# Autodesk Inventor assembly: СБ_Лицевой лист
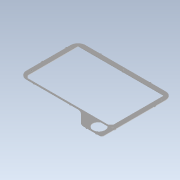
[picture p0: Inventor's stored thumbnail of the model, 180x180]
Saved by Autodesk Inventor 2021.2 (Build 252289000, 289)
## iProperties
Created: 2022-12-06
Part Number: СБ_Лицевой лист
Document SubType Name: Assembly
Designer: Королев В. В.
Mass: 46.2815 g
Surface Area: 491.583 cm^2
Volume: 42.8372 cm^3
Density: 1.0804 g/cm^3
Author: Королев В. В.
## Documents named in this file (3)
- C:\Users\Voodoo\Documents\Inventor\АБТ_Инфотабло\СБ_Лицевой лист.iam
- C:\Users\Voodoo\Documents\Inventor\АБТ_Инфотабло\Лицевой лист.ipt
- C:\Users\Voodoo\Documents\Inventor\АБТ_Инфотабло\Вытяжная заклепка_Р-Ш-М3-Ум.ipt
## Components (6 placed, 2 different names)
1. Лицевой лист:1
2. Вытяжная заклепка_Р-Ш-М3-Ум:1
3. Вытяжная заклепка_Р-Ш-М3-Ум:2
4. Вытяжная заклепка_Р-Ш-М3-Ум:3
5. Вытяжная заклепка_Р-Ш-М3-Ум:4
6. Вытяжная заклепка_Р-Ш-М3-Ум:5
## Relationships (5: Insert 5)
- [Insert]: Лицевой лист:1 ↔ Вытяжная заклепка_Р-Ш-М3-Ум:3
- [Insert]: Лицевой лист:1 ↔ Вытяжная заклепка_Р-Ш-М3-Ум:2
- [Insert]: Лицевой лист:1 ↔ Вытяжная заклепка_Р-Ш-М3-Ум:5
- [Insert]: Лицевой лист:1 ↔ Вытяжная заклепка_Р-Ш-М3-Ум:1
- [Insert]: Лицевой лист:1 ↔ Вытяжная заклепка_Р-Ш-М3-Ум:4
